# Autodesk Inventor assembly: End_Effector
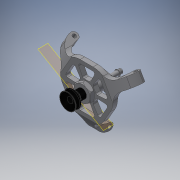
[picture p0: Inventor's stored thumbnail of the model, 180x180]
Saved by Autodesk Inventor 2019.4 (Build 234330000, 330)
## iProperties
Created: 2020-01-11
Part Number: End_Effector
Document SubType Name: Assembly
Designer: Jorian Bruslind
Author: Jorian Bruslind
## Documents named in this file (4)
- C:\Users\Jorian Bruslind\Documents\GitHub\ECE44x_Senior_Design\Design files\Delta Robot Arm\Inventor Files\Custom_Delta\End_Effector.iam
- C:\Users\Jorian Bruslind\Documents\GitHub\ECE44x_Senior_Design\Design files\Delta Robot Arm\Inventor Files\McMaster Files\5427A722_VACUUM CUP AND FITTING.ipt
- C:\Users\Jorian Bruslind\Documents\GitHub\ECE44x_Senior_Design\Design files\Delta Robot Arm\Inventor Files\Custom_Delta\End_EffectorV2.ipt
- C:\Users\Jorian Bruslind\Documents\GitHub\ECE44x_Senior_Design\Design files\Delta Robot Arm\Inventor Files\McMaster Files\5372K176_DURABLE NYLON EXTRA-GRIP BARBED TUBE FITTING.ipt
## Components (3 placed, 3 different names)
1. 5427A722_VACUUM CUP AND FITTING:1 — Mate:1, Mate:2, Mate:3
2. End_EffectorV2:1 — Mate:1, Mate:2, Mate:4
3. 5372K176_DURABLE NYLON EXTRA-GRIP BARBED TUBE FITTING:1 — Mate:3, Mate:4
## Relationships (4: Mate 4)
- Mate:1: 5427A722_VACUUM CUP AND FITTING:1 ↔ End_EffectorV2:1
- Mate:2: 5427A722_VACUUM CUP AND FITTING:1 ↔ End_EffectorV2:1
- Mate:3: 5427A722_VACUUM CUP AND FITTING:1 ↔ 5372K176_DURABLE NYLON EXTRA-GRIP BARBED TUBE FITTING:1
- Mate:4: End_EffectorV2:1 ↔ 5372K176_DURABLE NYLON EXTRA-GRIP BARBED TUBE FITTING:1
